# Autodesk Inventor assembly: assembled_v3
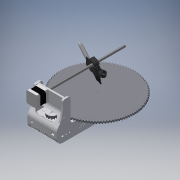
[picture p0: Inventor's stored thumbnail of the model, 180x180]
Saved by Autodesk Inventor 2016 (Build 200138000, 138)
## iProperties
Created: 2016-10-13
Part Number: assembled_v3
Document SubType Name: Assembly
Designer: brent
Author: brent
## Documents named in this file (6)
- C:\Users\brent\OneDrive\classes\desinv22\motorized_drawing_machine\assembled_v3.iam
- C:\Users\brent\OneDrive\classes\desinv22\motorized_drawing_machine\primary_v3.ipt
- C:\Users\brent\OneDrive\classes\desinv22\motorized_drawing_machine\offtheshelf\nema17_40mm_300mml.ipt
- C:\Users\brent\OneDrive\classes\desinv22\motorized_drawing_machine\offtheshelf\nema17_33mm.ipt
- C:\Users\brent\OneDrive\classes\desinv22\motorized_drawing_machine\offtheshelf\sharpie\Sharpie-Fine-Point.iam
- C:\Users\brent\OneDrive\classes\desinv22\motorized_drawing_machine\penholder_v3.ipt
## Components (5 placed, 5 different names)
1. primary_v3:1 — Mate:1, Mate:2, Mate:3, Mate:4, Mate:5, Mate:6, Mate:8
2. nema17_40mm_300mml:1 — Mate:2, Mate:3, Mate:4, Cylindrical:1
3. nema17_33mm:1 — Mate:5
4. Sharpie-Fine-Point:1 [sub-assembly] — Mate:7, Mate:8
5. penholder_v3:1 — Cylindrical:1, Mate:6, Mate:7
## Relationships (9: Mate 8, CylindricalJoint 1)
- Mate:1: primary_v3:1
- Mate:2: primary_v3:1 ↔ nema17_40mm_300mml:1
- Mate:3: primary_v3:1 ↔ nema17_40mm_300mml:1
- Mate:4: primary_v3:1 ↔ nema17_40mm_300mml:1
- Mate:5: primary_v3:1 ↔ nema17_33mm:1
- Cylindrical:1: nema17_40mm_300mml:1 ↔ penholder_v3:1
- Mate:6: primary_v3:1 ↔ penholder_v3:1
- Mate:7: Sharpie-Fine-Point:1 ↔ penholder_v3:1
- Mate:8: primary_v3:1 ↔ Sharpie-Fine-Point:1
